# Autodesk Inventor assembly: SliderAssembly
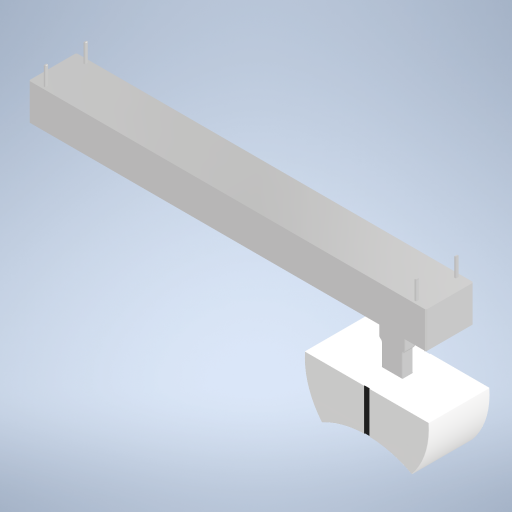
[picture p0: Inventor's stored thumbnail of the model, 512x512]
Saved by Autodesk Inventor 2023 (Build 270158000, 158)
## iProperties
Created: 2024-03-19
Part Number: SliderAssembly
Document SubType Name: Assembly
Designer: noname
Author: noname
## Documents named in this file (4)
- C:\Users\noname\Documents\GitHub\AudMix\3dModels\Slider\SliderAssembly.iam
- C:\Users\noname\Documents\GitHub\AudMix\3dModels\Slider\Body.ipt
- C:\Users\noname\Documents\GitHub\AudMix\3dModels\Slider\Cup.ipt
- C:\Users\noname\Documents\GitHub\AudMix\3dModels\Slider\Slider.ipt
## Components (3 placed, 3 different names)
1. Body:1 — Mate:1, Mate:2, Mate:3, Flush:1
2. Cup:1 — Mate:5, Mate:6, Flush:1
3. Slider:1 — Mate:1, Mate:2, Mate:3, Mate:5, Mate:6
## Relationships (6: Mate 5, Flush 1)
- Mate:1: Body:1 ↔ Slider:1
- Mate:2: Body:1 ↔ Slider:1
- Mate:3: Body:1 ↔ Slider:1
- Mate:5: Cup:1 ↔ Slider:1
- Mate:6: Cup:1 ↔ Slider:1
- Flush:1 (17 mm): Body:1 ↔ Cup:1
